# Autodesk Inventor assembly: Microswitch - Omron SS-01GL2-E
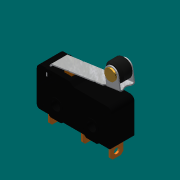
[picture p0: Inventor's stored thumbnail of the model, 180x180]
Saved by Autodesk Inventor 2016 (Build 200138000, 138)
## iProperties
Created: 2012-05-23
Document SubType Name: Assembly
Designer: sdarley
Project: Microswitch - Omron SS-01GL2-E
Catalog Web Link: http://australia.rs-online.com/web/p/microswitches/6822629/
Description: Microswitch - Omron SS-01GL2-E
Vendor: Omron
Stock Number: SS-01GL2-E
Author: sdarley
Title: Microswitch - Omron SS-01GL2-E
Revision Number: 1
## Documents named in this file (7)
- C:\Users\Sawaiz\Documents\data\projects\cncBlackBox\microswitch\microswitch.iam
- C:\Users\Sawaiz\Documents\data\projects\cncBlackBox\microswitch\housing.ipt
- C:\Users\Sawaiz\Documents\data\projects\cncBlackBox\microswitch\contact.ipt
- C:\Users\Sawaiz\Documents\data\projects\cncBlackBox\microswitch\button.ipt
- C:\Users\Sawaiz\Documents\data\projects\cncBlackBox\microswitch\springLever.ipt
- C:\Users\Sawaiz\Documents\data\projects\cncBlackBox\microswitch\rollerPin.ipt
- C:\Users\Sawaiz\Documents\data\projects\cncBlackBox\microswitch\roller.ipt
## Components (8 placed, 6 different names)
1. housing:1 — Flush:1, Flush:2, Flush:3, Flush:4, Mate:1, Flush:5, Mate:2, Mate:3, Mate:4, Mate:5, Flush:8, Mate:6, Mate:7, Flush:9, Mate:8, Flush:10, Mate:11
2. button:1 — Flush:8, Mate:6, Mate:7
3. springLever:1 — Flush:9, Mate:8, Flush:10, Flush:11, Mate:9
4. rollerPin:1 — Flush:11, Mate:9, Mate:10
5. roller:1 — Mate:10, Mate:11
6. contact:1 — Flush:4, Mate:1, Flush:5, Flush:6
7. contact:2 — Mate:3, Mate:4, Flush:6, Flush:7
8. contact:3 — Mate:2, Mate:5, Flush:7
## Relationships (22: Flush 11, Mate 11)
- Flush:1: housing:1
- Flush:2: housing:1
- Flush:3: housing:1
- Flush:4: housing:1 ↔ contact:1
- Mate:1: housing:1 ↔ contact:1
- Flush:5 (-1.6 mm): housing:1 ↔ contact:1
- Mate:2: housing:1 ↔ contact:3
- Mate:3: housing:1 ↔ contact:2
- Mate:4: housing:1 ↔ contact:2
- Mate:5: housing:1 ↔ contact:3
- Flush:6 (8.8 mm): contact:1 ↔ contact:2
- Flush:7 (7.3 mm): contact:2 ↔ contact:3
- Flush:8: housing:1 ↔ button:1
- Mate:6: housing:1 ↔ button:1
- Mate:7: housing:1 ↔ button:1
- Flush:9: housing:1 ↔ springLever:1
- Mate:8: housing:1 ↔ springLever:1
- Flush:10: housing:1 ↔ springLever:1
- Flush:11: springLever:1 ↔ rollerPin:1
- Mate:9: springLever:1 ↔ rollerPin:1
- Mate:10: rollerPin:1 ↔ roller:1
- Mate:11: housing:1 ↔ roller:1
